# Autodesk Inventor assembly: Assembly1
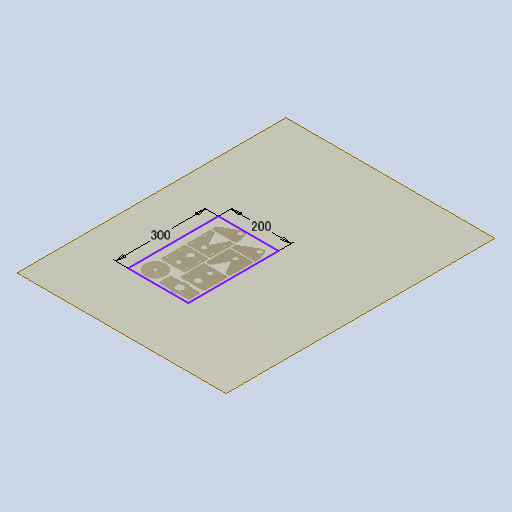
[picture p0: Inventor's stored thumbnail of the model, 512x512]
Saved by Autodesk Inventor 2025.1 (Build 291241000, 241)
## iProperties
Created: 2024-11-30
Part Number: Assembly1
Document SubType Name: Assembly
Designer: haruy
Author: haruy
## Documents named in this file (8)
- C:\Users\haruy\Documents\ロボコン\NHK2025\cad\cnc\Assembly1.iam
- C:\Users\haruy\Documents\ロボコン\NHK2025\cad\nagahisa\hand\grab\hand-grab-v3-Plate-ASP_F.ipt
- C:\Users\haruy\Documents\ロボコン\NHK2025\cad\nagahisa\hand\grab\hand-grab-v1-MDF-air-Base.ipt
- C:\Users\haruy\Documents\ロボコン\NHK2025\cad\nagahisa\ball_loading\ball_loading_v1_Plate_left_up_F.ipt
- C:\Users\haruy\Documents\ロボコン\NHK2025\cad\nagahisa\ball_loading\ball_loading_v1_Plate_right_down_R_F.ipt
- C:\Users\haruy\Documents\ロボコン\NHK2025\cad\nagahisa\ball_loading\ball_loading_v1_Plate_left_down_R_F.ipt
- C:\Users\haruy\Documents\ロボコン\NHK2025\cad\nagahisa\ball_loading\ball_loading_v1_Plate_right_down_M_F.ipt
- C:\Users\haruy\Documents\ロボコン\NHK2025\cad\nagahisa\ball_loading\ball_loading_v1_Plate_left_down_M_F.ipt
## Components (8 placed, 7 different names)
1. hand-grab-v3-Plate-ASP_F:1 — フラッシュ:3, フラッシュ:25
2. hand-grab-v1-MDF-air-Base:1 — フラッシュ:2
3. ball_loading_v1_Plate_left_up_F:1 — フラッシュ:19, フラッシュ:28, メイト:6
4. ball_loading_v1_Plate_left_up_F:2 — フラッシュ:20, フラッシュ:27, メイト:5
5. ball_loading_v1_Plate_right_down_R_F:1 — フラッシュ:21, メイト:3, メイト:4, フラッシュ:28, メイト:6
6. ball_loading_v1_Plate_left_down_R_F:1 — フラッシュ:22, フラッシュ:26, メイト:1, メイト:3, フラッシュ:27, メイト:5
7. ball_loading_v1_Plate_right_down_M_F:1 — フラッシュ:23, メイト:2, メイト:4
8. ball_loading_v1_Plate_left_down_M_F:1 — フラッシュ:24, フラッシュ:25, フラッシュ:26, メイト:1, メイト:2
## Relationships (18: Flush 12, Mate 6)
- フラッシュ:2 [Flush]: hand-grab-v1-MDF-air-Base:1
- フラッシュ:3 [Flush]: hand-grab-v3-Plate-ASP_F:1
- フラッシュ:19 [Flush]: ball_loading_v1_Plate_left_up_F:1
- フラッシュ:20 [Flush]: ball_loading_v1_Plate_left_up_F:2
- フラッシュ:21 [Flush]: ball_loading_v1_Plate_right_down_R_F:1
- フラッシュ:22 [Flush]: ball_loading_v1_Plate_left_down_R_F:1
- フラッシュ:23 [Flush]: ball_loading_v1_Plate_right_down_M_F:1
- フラッシュ:24 [Flush]: ball_loading_v1_Plate_left_down_M_F:1
- フラッシュ:25 [Flush]: hand-grab-v3-Plate-ASP_F:1 ↔ ball_loading_v1_Plate_left_down_M_F:1
- フラッシュ:26 [Flush]: ball_loading_v1_Plate_left_down_R_F:1 ↔ ball_loading_v1_Plate_left_down_M_F:1
- メイト:1 [Mate] (5 mm): ball_loading_v1_Plate_left_down_R_F:1 ↔ ball_loading_v1_Plate_left_down_M_F:1
- メイト:2 [Mate] (5 mm): ball_loading_v1_Plate_right_down_M_F:1 ↔ ball_loading_v1_Plate_left_down_M_F:1
- メイト:3 [Mate] (5 mm): ball_loading_v1_Plate_right_down_R_F:1 ↔ ball_loading_v1_Plate_left_down_R_F:1
- メイト:4 [Mate] (5 mm): ball_loading_v1_Plate_right_down_R_F:1 ↔ ball_loading_v1_Plate_right_down_M_F:1
- フラッシュ:27 [Flush]: ball_loading_v1_Plate_left_up_F:2 ↔ ball_loading_v1_Plate_left_down_R_F:1
- メイト:5 [Mate] (5 mm): ball_loading_v1_Plate_left_up_F:2 ↔ ball_loading_v1_Plate_left_down_R_F:1
- フラッシュ:28 [Flush]: ball_loading_v1_Plate_left_up_F:1 ↔ ball_loading_v1_Plate_right_down_R_F:1
- メイト:6 [Mate] (5 mm): ball_loading_v1_Plate_left_up_F:1 ↔ ball_loading_v1_Plate_right_down_R_F:1
